# Autodesk Inventor assembly: BBot
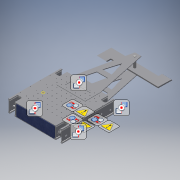
[picture p0: Inventor's stored thumbnail of the model, 180x180]
Saved by Autodesk Inventor 2017 (Build 210142000, 142)
## iProperties
Created: 2016-10-21
Part Number: BBot
Document SubType Name: Assembly
Designer: aesen
Author: aesen
## Documents named in this file (13)
- C:\Users\aesen\Design\for assambly\BBot.iam
- C:\Users\aesen\Design\for assambly\1021topDT.ipt
- C:\Users\aesen\Design\for assambly\1021sidemotor.ipt
- C:\Users\aesen\Design\updated drive train\gearsystem1.iam
- C:\Users\aesen\Design\updated drive train\gearsystem2.iam
- C:\Users\aesen\Design\updated drive train\gearsystem3.iam
- C:\Users\aesen\Design\for assambly\1021sidenomotorN.ipt
- C:\Users\aesen\Design\for assambly\1021TopP.ipt
- C:\Users\aesen\Design\for assambly\W1support.ipt
- C:\Users\aesen\Design\for assambly\Blunt_Blade.ipt
- C:\Users\aesen\Design\for assambly\BBot\Design Accelerator\Shaft1.iam
- C:\Users\aesen\Design\for assambly\backpanel.ipt
- C:\Users\aesen\Design\for assambly\frontpannel.ipt
## Components (26 placed, 12 different names)
1. 1021topDT:7 — Mate:5, Mate:6, Mate:12, Mate:13, Mate:14
2. 1021topDT:8 — Mate:3, Mate:4, Mate:7, Mate:8, Mate:17, Mate:18
3. gearsystem3:1 [sub-assembly] — Insert:2, Insert:3, Rotation:2, Rotation:3, Rotation:11
4. gearsystem3:2 [sub-assembly] — Insert:6, Insert:7, Rotation:6, Rotation:7
5. gearsystem2:1 [sub-assembly] — Insert:3, Insert:4, Rotation:3, Rotation:4
6. gearsystem2:2 [sub-assembly] — Insert:5, Insert:6, Rotation:7, Rotation:8
7. gearsystem2:3 [sub-assembly] — Insert:1, Insert:2, Rotation:1, Rotation:2
8. gearsystem2:4 [sub-assembly] — Insert:7, Insert:8, Rotation:5, Rotation:6
9. gearsystem1:1 [sub-assembly] — Insert:1, Rotation:1
10. gearsystem1:2 [sub-assembly] — Insert:8, Rotation:5
11. gearsystem1:3 [sub-assembly] — Insert:4, Rotation:4
12. gearsystem1:4 [sub-assembly] — Insert:5, Rotation:8, Rotation:12
13. 1021topDT:9 — Mate:1, Mate:2, Mate:15, Mate:16
14. 1021sidenomotorN:1 — Mate:1, Mate:2, Mate:5, Mate:6, Mate:14, Rotation:12
15. 1021sidenomotorN:2 — Mate:3, Mate:4, Mate:9, Mate:10, Rotation:11
16. 1021topDT:10 — Mate:9, Mate:10, Mate:11, Mate:19, Mate:20
17. 1021sidemotor:1 — Mate:7, Mate:8, Mate:11
18. 1021sidemotor:2 — Mate:12, Mate:13
19. W1support:1 — Rotation:13, Insert:10
20. W1support:2 — Rotation:14, Rotation:15
21. 1021TopP:1 — Mate:15, Mate:16, Mate:17, Mate:18, Rotation:14, Rotation:15, Flush:1, Flush:2, Flush:3, Flush:5, Flush:6, Flush:8, Mate:21
22. 1021TopP:2 — Mate:19, Mate:20, Rotation:13, Flush:4, Flush:7
23. Blunt_Blade:1 — Insert:9
24. Shaft:1 [sub-assembly] — Insert:9, Insert:10
25. backpanel:1 — Flush:1, Flush:2, Flush:3, Flush:4
26. frontpannel:1 — Flush:5, Flush:6, Flush:7, Flush:8, Mate:21
## Relationships (52: Mate 21, RelateRotation 13, Insert 10, Flush 8)
- Insert:1 (-38.1 mm): gearsystem2:3 ↔ gearsystem1:1
- Insert:2 (-38.1 mm): gearsystem3:1 ↔ gearsystem2:3
- Insert:3 (-38.1 mm): gearsystem3:1 ↔ gearsystem2:1
- Insert:4 (-27.94 mm): gearsystem2:1 ↔ gearsystem1:3
- Insert:5 (-38.1 mm): gearsystem2:2 ↔ gearsystem1:4
- Insert:6 (-38.1 mm): gearsystem3:2 ↔ gearsystem2:2
- Insert:7 (-38.1 mm): gearsystem3:2 ↔ gearsystem2:4
- Insert:8 (-38.1 mm): gearsystem2:4 ↔ gearsystem1:2
- Rotation:1 [RelateRotation] (1 ul): gearsystem2:3 ↔ gearsystem1:1
- Rotation:2 [RelateRotation] (1 ul): gearsystem3:1 ↔ gearsystem2:3
- Rotation:3 [RelateRotation] (1 ul): gearsystem3:1 ↔ gearsystem2:1
- Rotation:4 [RelateRotation] (1 ul): gearsystem2:1 ↔ gearsystem1:3
- Rotation:5 [RelateRotation] (1 ul): gearsystem2:4 ↔ gearsystem1:2
- Rotation:6 [RelateRotation] (1 ul): gearsystem3:2 ↔ gearsystem2:4
- Rotation:7 [RelateRotation] (1 ul): gearsystem3:2 ↔ gearsystem2:2
- Rotation:8 [RelateRotation] (1 ul): gearsystem2:2 ↔ gearsystem1:4
- Mate:1: 1021topDT:9 ↔ 1021sidenomotorN:1
- Mate:2: 1021topDT:9 ↔ 1021sidenomotorN:1
- Mate:3: 1021topDT:8 ↔ 1021sidenomotorN:2
- Mate:4: 1021topDT:8 ↔ 1021sidenomotorN:2
- Mate:5: 1021topDT:7 ↔ 1021sidenomotorN:1
- Mate:6: 1021topDT:7 ↔ 1021sidenomotorN:1
- Mate:7: 1021topDT:8 ↔ 1021sidemotor:1
- Mate:8: 1021topDT:8 ↔ 1021sidemotor:1
- Mate:9: 1021sidenomotorN:2 ↔ 1021topDT:10
- Mate:10: 1021sidenomotorN:2 ↔ 1021topDT:10
- Mate:11: 1021topDT:10 ↔ 1021sidemotor:1
- Mate:12: 1021topDT:7 ↔ 1021sidemotor:2
- Mate:13: 1021topDT:7 ↔ 1021sidemotor:2
- Mate:14: 1021topDT:7 ↔ 1021sidenomotorN:1
- Rotation:11 [RelateRotation] (1 ul): gearsystem3:1 ↔ 1021sidenomotorN:2
- Rotation:12 [RelateRotation] (1 ul): gearsystem1:4 ↔ 1021sidenomotorN:1
- Mate:15: 1021topDT:9 ↔ 1021TopP:1
- Mate:16: 1021topDT:9 ↔ 1021TopP:1
- Mate:17: 1021topDT:8 ↔ 1021TopP:1
- Mate:18: 1021topDT:8 ↔ 1021TopP:1
- Mate:19: 1021topDT:10 ↔ 1021TopP:2
- Mate:20: 1021topDT:10 ↔ 1021TopP:2
- Rotation:13 [RelateRotation] (1 ul): W1support:1 ↔ 1021TopP:2
- Rotation:14 [RelateRotation] (1 ul): W1support:2 ↔ 1021TopP:1
- Rotation:15 [RelateRotation]: W1support:2 ↔ 1021TopP:1
- Insert:9 (-114.3 mm): Blunt_Blade:1 ↔ Shaft:1
- Insert:10 (-10.16 mm): W1support:1 ↔ Shaft:1
- Flush:1: 1021TopP:1 ↔ backpanel:1
- Flush:2: 1021TopP:1 ↔ backpanel:1
- Flush:3: 1021TopP:1 ↔ backpanel:1
- Flush:4: 1021TopP:2 ↔ backpanel:1
- Flush:5: 1021TopP:1 ↔ frontpannel:1
- Flush:6: 1021TopP:1 ↔ frontpannel:1
- Flush:7: 1021TopP:2 ↔ frontpannel:1
- Flush:8: 1021TopP:1 ↔ frontpannel:1
- Mate:21: 1021TopP:1 ↔ frontpannel:1
